# Autodesk Inventor assembly: puk_centered
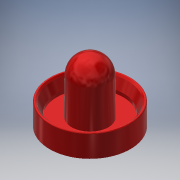
[picture p0: Inventor's stored thumbnail of the model, 180x180]
Saved by Autodesk Inventor 2019.3 (Build 233278000, 278)
## iProperties
Created: 2020-12-03
Part Number: puk_centered
Material: Generisch
Document SubType Name: Assembly
Designer: Nicolas Frick
Author: Nicolas Frick
## Documents named in this file (3)
- C:\Users\Nicolas Frick\Sync\OneDrive\airhockeybot\mechanical_design\common_cad_parts\sim_models\puk_centered.iam
- C:\Users\Nicolas Frick\Sync\OneDrive\airhockeybot\mechanical_design\inventor\bat.ipt
- C:\Users\Nicolas Frick\Sync\OneDrive\airhockeybot\mechanical_design\inventor\bat_handle.ipt
## Components (2 placed, 2 different names)
1. bat:1 — Passend:1, Passend:2, Passend:3, Passend:4
2. bat_handle:1 — Passend:2, Passend:3
## Relationships (4: Mate 4)
- Passend:1 [Mate]: bat:1
- Passend:2 [Mate]: bat:1 ↔ bat_handle:1
- Passend:3 [Mate]: bat:1 ↔ bat_handle:1
- Passend:4 [Mate]: bat:1
